# Autodesk Inventor assembly: Assembly
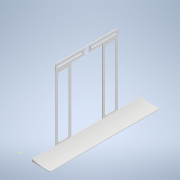
[picture p0: Inventor's stored thumbnail of the model, 180x180]
Saved by Autodesk Inventor 2020.2 (Build 242310000, 310)
## iProperties
Created: 2020-05-07
Part Number: Assembly
Document SubType Name: Assembly
Designer: Amaan Khalid
Author: Amaan Khalid
## Documents named in this file (3)
- C:\Users\Amaan Khalid\Desktop\My projects\Benq Pen Holder\Assembly.iam
- C:\Users\Amaan Khalid\Desktop\My projects\Benq Pen Holder\Part On Monitor.ipt
- C:\Users\Amaan Khalid\Desktop\My projects\Benq Pen Holder\Pen Holder.ipt
## Components (2 placed, 2 different names)
1. Part On Monitor:1 — Mate:1, Mate:2
2. Pen Holder:1 — Mate:1, Mate:2
## Relationships (2: Mate 2)
- Mate:1: Part On Monitor:1 ↔ Pen Holder:1
- Mate:2: Part On Monitor:1 ↔ Pen Holder:1
